# Autodesk Inventor assembly: ASY PNS 760 elbow
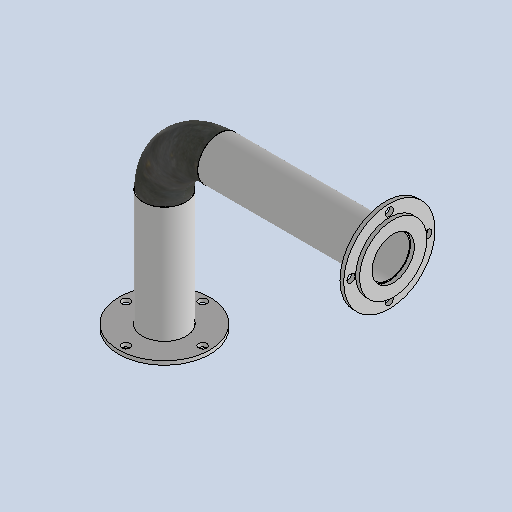
[picture p0: Inventor's stored thumbnail of the model, 512x512]
Saved by Autodesk Inventor 2025.1 (Build 291241020, 241B)
## iProperties
Created: 2025-07-04
Part Number: ASY PNS 760 elbow
Document SubType Name: Assembly
Designer: user
Author: user
## Documents named in this file (6)
- C:\Users\user\YandexDisk-badmisterfox\home pc\Inventor\PNS-Panaevsk\Filter D1200\ASY PNS 760 elbow.iam
- C:\Users\user\YandexDisk-badmisterfox\home pc\Inventor\PNS-Panaevsk\CC\en-US\JIS B 2312 90 (2)\JIS B 2312 90 Deg Long Elbow Steel 80A x Sch 40.ipt
- C:\Users\user\YandexDisk-badmisterfox\home pc\Inventor\PNS-Panaevsk\Filter D1200\PNS 755 FDS tube.ipt
- C:\Users\user\YandexDisk-badmisterfox\home pc\Inventor\PNS-Panaevsk\Filter D1200\PNS 734 FDS flange DN90.ipt
- C:\Users\user\YandexDisk-badmisterfox\home pc\Inventor\PNS-Panaevsk\Filter D1200\PNS 735 FDS free flange DN90.ipt
- C:\Users\user\YandexDisk-badmisterfox\home pc\Inventor\PNS-Panaevsk\Filter D1200\PNS 756 FDS tube.ipt
## Components (7 placed, 5 different names)
1. JIS B 2312 90 Deg Long Elbow Steel 80A x Sch 40:1
2. PNS 755 FDS tube:1
3. PNS 734 FDS flange DN90:1
4. PNS 735 FDS free flange DN90:1
5. PNS 756 FDS tube:1
6. PNS 734 FDS flange DN90:2
7. PNS 735 FDS free flange DN90:2
## Relationships (6: WeldJoint 6)
- [WeldJoint]: PNS 755 FDS tube:1 ↔ PNS 735 FDS free flange DN90:1
- [WeldJoint]: PNS 755 FDS tube:1 ↔ PNS 734 FDS flange DN90:1
- [WeldJoint]: JIS B 2312 90 Deg Long Elbow Steel 80A x Sch 40:1 ↔ PNS 755 FDS tube:1
- [WeldJoint]: JIS B 2312 90 Deg Long Elbow Steel 80A x Sch 40:1 ↔ PNS 756 FDS tube:1
- [WeldJoint]: PNS 756 FDS tube:1 ↔ PNS 735 FDS free flange DN90:2
- [WeldJoint]: PNS 734 FDS flange DN90:2 ↔ PNS 735 FDS free flange DN90:2
